# Autodesk Inventor assembly: motor_antigravity_4004_custom_shaft
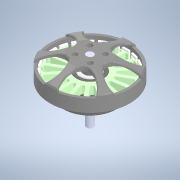
[picture p0: Inventor's stored thumbnail of the model, 180x180]
Saved by Autodesk Inventor 2022.2 (Build 262287030, 287C)
## iProperties
Created: 2016-08-15
Part Number: motor_antigravity_4004_custom_shaft
Document SubType Name: Assembly
Designer: Jochen
Sending System: SolidWorks 2017
Last Author: Felix
Last Saved: 2021-02-23
Author: Jochen
## Documents named in this file (5)
- D:\Projects\Lisbeth\CAD\Common\Motor\motor_antigravity_4004_custom_shaft.iam
- D:\Projects\Lisbeth\CAD\Common\Motor\motor_antigravity_4004_stator.ipt
- D:\Projects\Lisbeth\CAD\Common\Motor\motor_antigravity_4004_rotor.ipt
- D:\Projects\Lisbeth\CAD\Common\Motor\motor_antigravity_4004_custom_shaft.ipt
- D:\Projects\Lisbeth\CAD\Common\Motor\motor_antigravity_4004_brass_spacer.ipt
## Components (4 placed, 4 different names)
1. motor_antigravity_4004_stator:1
2. motor_antigravity_4004_rotor:1 — Mate:1, Mate:2
3. motor_antigravity_4004_custom_shaft:1 — Mate:1, Mate:2
4. motor_antigravity_4004_brass_spacer:1
## Relationships (2: Mate 2)
- Mate:1: motor_antigravity_4004_rotor:1 ↔ motor_antigravity_4004_custom_shaft:1
- Mate:2: motor_antigravity_4004_rotor:1 ↔ motor_antigravity_4004_custom_shaft:1
